# Autodesk Inventor assembly: FullAssembly0.1
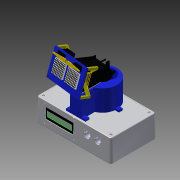
[picture p0: Inventor's stored thumbnail of the model, 180x180]
Saved by Autodesk Inventor 2015 (Build 190159000, 159)
## iProperties
Created: 2015-03-06
Part Number: FullAssembly0.1
Document SubType Name: Assembly
Designer: ChristopherEvan
Author: ChristopherEvan
## Documents named in this file (5)
- C:\Users\ChristopherEvan\Documents\Inventor\MAKE\FullAssembly0.1.iam
- C:\Users\ChristopherEvan\Documents\Inventor\MAKE\Enclosure\Enclosure.iam
- C:\Users\ChristopherEvan\Documents\Inventor\MAKE\Enclosure\ProxSensor\hc-sr04.iam
- C:\Users\ChristopherEvan\Documents\Inventor\MAKE\Enclosure\LCD\LCD_with_bracket.iam
- C:\Users\ChristopherEvan\Documents\Inventor\MAKE\Head\Head.iam
## Components (4 placed, 4 different names)
1. Enclosure:1 [sub-assembly] — Mate:1, Mate:2, Mate:3, Mate:4
2. hc-sr04:1 [sub-assembly] — Mate:1
3. LCD_with_bracket:1 [sub-assembly] — Mate:2
4. Head:1 [sub-assembly] — Mate:3, Mate:4, Angle:1
## Relationships (5: Mate 4, Angle 1)
- Mate:1: Enclosure:1 ↔ hc-sr04:1
- Mate:2: Enclosure:1 ↔ LCD_with_bracket:1
- Mate:3: Enclosure:1 ↔ Head:1
- Mate:4: Enclosure:1 ↔ Head:1
- Angle:1 (0 deg): Head:1
